# Autodesk Inventor assembly: Motors with Screws
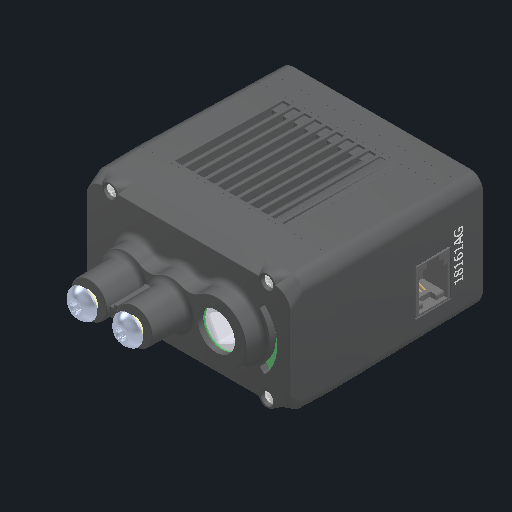
[picture p0: Inventor's stored thumbnail of the model, 512x512]
Saved by Autodesk Inventor 2025 (Build 290162000, 162)
## iProperties
Created: 2022-08-18
Part Number: Motors with Screws
Document SubType Name: Assembly
Designer: ylu12
Author: ylu12
## Documents named in this file (10)
- D:\vex_robotics_high_stakes\hardware\cad\robpros_cad_lib\Electronics\Motors with Screws.iam
- D:\vex_robotics_high_stakes\hardware\cad\robpros_cad_lib\Electronics\V5 Motor.ipt
- D:\vex_robotics_high_stakes\hardware\cad\robpros_cad_lib\Structure\Hardware\Screw Steel - Hex\SScrew Hex Smooth .500.ipt
- C:\Users\ylu12\Documents\GitHub\VEX-CAD-Inventor\Structure\Hardware\Screw Steel - Hex.ipt
- D:\vex_robotics_high_stakes\hardware\cad\robpros_cad_lib\Structure\Hardware\Screw Steel - Star\SScrew Star Smooth .500.ipt
- C:\Users\ylu12\Documents\GitHub\VEX-CAD-Inventor\Structure\Hardware\Screw Steel - Star.ipt
- AluM-HexS.iam
- AluM-StarS.iam
- SteelM-HexS.iam
- SteelM-StarS.iam
## Components (5 placed, 3 different names)
1. V5 Motor:1 — Insert:1, Insert:2
2. SScrew Hex Smooth .500:1 — Insert:1, Insert:3
3. SScrew Hex Smooth .500:2 — Insert:2, Insert:4
4. SScrew Star Smooth .500:1 — Insert:4
5. SScrew Star Smooth .500:2 — Insert:3
## Relationships (4: Insert 4)
- Insert:1: V5 Motor:1 ↔ SScrew Hex Smooth .500:1
- Insert:2: V5 Motor:1 ↔ SScrew Hex Smooth .500:2
- Insert:3: SScrew Hex Smooth .500:1 ↔ SScrew Star Smooth .500:2
- Insert:4: SScrew Hex Smooth .500:2 ↔ SScrew Star Smooth .500:1
## Named parameters: Thickness = 1.19063 mm
